# Autodesk Inventor assembly: ROBOT_1_3
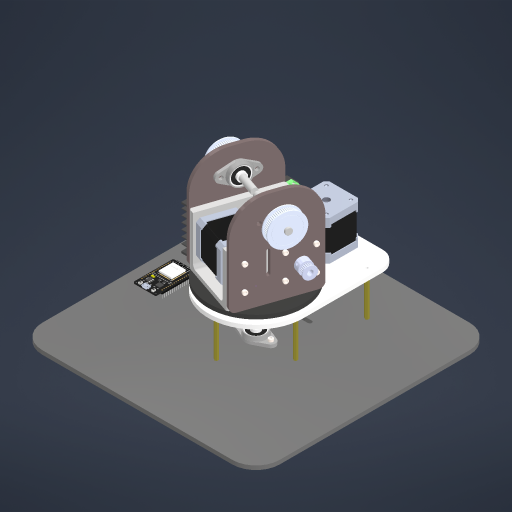
[picture p0: Inventor's stored thumbnail of the model, 512x512]
Saved by Autodesk Inventor 2023 (Build 270158000, 158)
## iProperties
Created: 2023-09-06
Part Number: ROBOT_1_3
Document SubType Name: Assembly
Designer: philo
Sending System: Autodesk Inventor 2023
Preprocessor: ST-DEVELOPER v19
Title: C:\Users\philo\OneDrive\Desktop\HK1-2024\TT ROBOT\3DVer2\ROBOT_1_2.stp
Author: philo
## Documents named in this file (23)
- C:\Users\philo\OneDrive\Desktop\HK1-2024\TT ROBOT\3DVer2\3DVer2\ROBOT_1_3.iam
- C:\Users\philo\OneDrive\Desktop\HK1-2024\TT ROBOT\3DVer2\3DVer2\DeRobot.ipt
- C:\Users\philo\OneDrive\Desktop\HK1-2024\TT ROBOT\3DVer2\3DVer2\Detron.ipt
- C:\Users\philo\OneDrive\Desktop\HK1-2024\TT ROBOT\3DVer2\3DVer2\goidoObi.ipt
- C:\Users\philo\OneDrive\Desktop\HK1-2024\TT ROBOT\3DVer2\3DVer2\truday.ipt
- C:\Users\philo\OneDrive\Desktop\HK1-2024\TT ROBOT\3DVer2\3DVer2\gt2_60teeth.iam
- C:\Users\philo\OneDrive\Desktop\HK1-2024\TT ROBOT\3DVer2\3DVer2\STEP MOTOR NEMA 17.ipt
- C:\Users\philo\OneDrive\Desktop\HK1-2024\TT ROBOT\3DVer2\3DVer2\GT2 Pulley 20 Tooth (ID6mm).ipt
- C:\Users\philo\OneDrive\Desktop\HK1-2024\TT ROBOT\3DVer2\3DVer2\M3 x 5mm.ipt
- C:\Users\philo\OneDrive\Desktop\HK1-2024\TT ROBOT\3DVer2\3DVer2\Diaquay.ipt
- C:\Users\philo\OneDrive\Desktop\HK1-2024\TT ROBOT\3DVer2\3DVer2\Tb6600.ipt
- C:\Users\philo\OneDrive\Desktop\HK1-2024\TT ROBOT\3DVer2\3DVer2\ESP-WROOM32.iam
- C:\Users\philo\OneDrive\Desktop\HK1-2024\TT ROBOT\3DVer2\3DVer2\codinhtruc.ipt
- C:\Users\philo\OneDrive\Desktop\HK1-2024\TT ROBOT\3DVer2\3DVer2\daydai.ipt
- C:\Users\philo\OneDrive\Desktop\HK1-2024\TT ROBOT\3DVer2\3DVer2\gt2smooth.ipt
- C:\Users\philo\OneDrive\Desktop\HK1-2024\TT ROBOT\3DVer2\3DVer2\trudong5mm.ipt
- C:\Users\philo\OneDrive\Desktop\HK1-2024\TT ROBOT\3DVer2\3DVer2\trucdogt2.ipt
- C:\Users\philo\OneDrive\Desktop\HK1-2024\TT ROBOT\3DVer2\3DVer2\HALL.ipt
- C:\Users\philo\OneDrive\Desktop\HK1-2024\TT ROBOT\3DVer2\3DVer2\namcham.ipt
- C:\Users\philo\OneDrive\Desktop\HK1-2024\TT ROBOT\3DVer2\3DVer2\Tamop1.ipt
- C:\Users\philo\OneDrive\Desktop\HK1-2024\TT ROBOT\3DVer2\3DVer2\60pitch pulley GT2 6mm ASSEMBLY.iam
- C:\Users\philo\OneDrive\Desktop\HK1-2024\TT ROBOT\3DVer2\3DVer2\truc8mm.ipt
- C:\Users\philo\OneDrive\Desktop\HK1-2024\TT ROBOT\3DVer2\3DVer2\giulink2.ipt
## Components (56 placed, 22 different names)
1. DeRobot:1
2. Detron:1 — Mate:33
3. goidoObi:1
4. goidoObi:2
5. truday:1 — Mate:32
6. gt2_60teeth:1 [sub-assembly]
7. STEP MOTOR NEMA 17:1
8. GT2 Pulley 20 Tooth (ID6mm):1
9. M3 x 5mm:1
10. M3 x 5mm:2
11. M3 x 5mm:3
12. M3 x 5mm:5
13. M3 x 5mm:6
14. M3 x 5mm:7
15. M3 x 5mm:8
16. Tb6600:1
17. Tb6600:2
18. ESP-WROOM32:1 [sub-assembly]
19. daydai:1
20. gt2smooth:1
21. trudong5mm:4
22. trudong5mm:5
23. trudong5mm:6
24. trudong5mm:8
25. trudong5mm:9
26. trucdogt2:1
27. HALL:1
28. M3 x 5mm:9 — Mate:38, Mate:56
29. M3 x 5mm:10 — Mate:39, Mate:58
30. M3 x 5mm:11 — Mate:37, Mate:60
31. M3 x 5mm:12 — Mate:40, Mate:57
32. M3 x 5mm:13 — Mate:41, Mate:61
33. M3 x 5mm:14 — Mate:42, Mate:59
34. M3 x 5mm:15 — Mate:43, Mate:52
35. M3 x 5mm:16 — Mate:45, Mate:51
36. M3 x 5mm:17 — Mate:46, Mate:54
37. M3 x 5mm:18 — Mate:44, Mate:50
38. M3 x 5mm:19 — Mate:47, Mate:53
39. M3 x 5mm:20 — Mate:48, Mate:55
40. gt2smooth:2 — Mate:49
41. giulink2:1 — Mate:63, Angle:3, Angle:4, Angle:5, Angle:6, Angle:7, Angle:8, Mate:64, Mate:65, Mate:67, Flush:4, Flush:5, Mate:68, Mate:69
42. Diaquay:1 — Mate:1, Mate:2, Mate:7, Mate:8, Mate:32, Mate:33, Mate:34, Angle:1, Angle:2, Flush:2, Mate:62, Flush:3, Angle:7
43. codinhtruc:2 — Mate:1, Mate:2, Mate:34, Mate:63
44. namcham:1 — Angle:2, Flush:2, Mate:62, Flush:3
45. STEP MOTOR NEMA 17:2 — Mate:27, Mate:28, Angle:6, Mate:66, Mate:67
46. STEP MOTOR NEMA 17:3 — Mate:26, Mate:30, Angle:5, Angle:8, Mate:64, Mate:65
47. Tamop1:1 — Mate:7, Mate:11, Mate:14, Mate:15, Mate:21, Flush:1, Mate:27, Mate:29, Mate:37, Mate:38, Mate:39, Mate:40, Mate:41, Mate:42, Mate:56, Mate:57, Mate:58, Mate:59, Mate:60, Mate:61, Angle:3, Mate:66, Flush:4, Mate:69
48. goidoObi:3 — Mate:11, Mate:14, Mate:15, Mate:18
49. GT2 Pulley 20 Tooth (ID6mm):2 — Mate:28, Mate:29
50. 60pitch pulley GT2 6mm ASSEMBLY:1 [sub-assembly] — Mate:21, Mate:22
51. Tamop1:2 — Mate:8, Mate:12, Mate:13, Mate:16, Mate:19, Mate:26, Mate:31, Angle:1, Mate:43, Mate:44, Mate:45, Mate:46, Mate:47, Mate:48, Mate:49, Mate:50, Mate:51, Mate:52, Mate:53, Mate:54, Mate:55, Angle:4, Flush:5, Mate:68
52. goidoObi:4 — Mate:12, Mate:13, Mate:16, Mate:17
53. GT2 Pulley 20 Tooth (ID6mm):3 — Mate:30, Mate:31
54. 60pitch pulley GT2 6mm ASSEMBLY:2 [sub-assembly] — Mate:19, Mate:20
55. truc8mm:1 — Mate:18, Mate:22, Mate:23, Flush:1
56. truc8mm:2 — Mate:17, Mate:20, Mate:23
## Relationships (72: Mate 59, Angle 8, Flush 5)
- Mate:1: Diaquay:1 ↔ codinhtruc:2
- Mate:2: Diaquay:1 ↔ codinhtruc:2
- Mate:7: Diaquay:1 ↔ Tamop1:1
- Mate:8: Diaquay:1 ↔ Tamop1:2
- Mate:11: Tamop1:1 ↔ goidoObi:3
- Mate:12: Tamop1:2 ↔ goidoObi:4
- Mate:13: Tamop1:2 ↔ goidoObi:4
- Mate:14: Tamop1:1 ↔ goidoObi:3
- Mate:15: Tamop1:1 ↔ goidoObi:3
- Mate:16: Tamop1:2 ↔ goidoObi:4
- Mate:17: goidoObi:4 ↔ truc8mm:2
- Mate:18: goidoObi:3 ↔ truc8mm:1
- Mate:19 (3 mm): Tamop1:2 ↔ 60pitch pulley GT2 6mm ASSEMBLY:2
- Mate:20: 60pitch pulley GT2 6mm ASSEMBLY:2 ↔ truc8mm:2
- Mate:21 (3 mm): Tamop1:1 ↔ 60pitch pulley GT2 6mm ASSEMBLY:1
- Mate:22: 60pitch pulley GT2 6mm ASSEMBLY:1 ↔ truc8mm:1
- Mate:23 (5 mm): truc8mm:1 ↔ truc8mm:2
- Flush:1 (-36 mm): Tamop1:1 ↔ truc8mm:1
- Mate:26: STEP MOTOR NEMA 17:3 ↔ Tamop1:2
- Mate:27: STEP MOTOR NEMA 17:2 ↔ Tamop1:1
- Mate:28: STEP MOTOR NEMA 17:2 ↔ GT2 Pulley 20 Tooth (ID6mm):2
- Mate:29 (3 mm): Tamop1:1 ↔ GT2 Pulley 20 Tooth (ID6mm):2
- Mate:30: STEP MOTOR NEMA 17:3 ↔ GT2 Pulley 20 Tooth (ID6mm):3
- Mate:31 (3 mm): Tamop1:2 ↔ GT2 Pulley 20 Tooth (ID6mm):3
- Mate:32: truday:1 ↔ Diaquay:1
- Mate:33 (6 mm): Detron:1 ↔ Diaquay:1
- Mate:34: Diaquay:1 ↔ codinhtruc:2
- Angle:1 (0 deg): Diaquay:1 ↔ Tamop1:2
- Angle:2 (0 deg): Diaquay:1 ↔ namcham:1
- Flush:2 (-60 mm): Diaquay:1 ↔ namcham:1
- Mate:37: M3 x 5mm:11 ↔ Tamop1:1
- Mate:38: M3 x 5mm:9 ↔ Tamop1:1
- Mate:39: M3 x 5mm:10 ↔ Tamop1:1
- Mate:40: M3 x 5mm:12 ↔ Tamop1:1
- Mate:41: M3 x 5mm:13 ↔ Tamop1:1
- Mate:42: M3 x 5mm:14 ↔ Tamop1:1
- Mate:43: M3 x 5mm:15 ↔ Tamop1:2
- Mate:44: M3 x 5mm:18 ↔ Tamop1:2
- Mate:45: M3 x 5mm:16 ↔ Tamop1:2
- Mate:46: M3 x 5mm:17 ↔ Tamop1:2
- Mate:47: M3 x 5mm:19 ↔ Tamop1:2
- Mate:48: M3 x 5mm:20 ↔ Tamop1:2
- Mate:49 (8 mm): gt2smooth:2 ↔ Tamop1:2
- Mate:50: M3 x 5mm:18 ↔ Tamop1:2
- Mate:51: M3 x 5mm:16 ↔ Tamop1:2
- Mate:52: M3 x 5mm:15 ↔ Tamop1:2
- Mate:53: M3 x 5mm:19 ↔ Tamop1:2
- Mate:54: M3 x 5mm:17 ↔ Tamop1:2
- Mate:55: M3 x 5mm:20 ↔ Tamop1:2
- Mate:56: M3 x 5mm:9 ↔ Tamop1:1
- Mate:57: M3 x 5mm:12 ↔ Tamop1:1
- Mate:58: M3 x 5mm:10 ↔ Tamop1:1
- Mate:59: M3 x 5mm:14 ↔ Tamop1:1
- Mate:60: M3 x 5mm:11 ↔ Tamop1:1
- Mate:61: M3 x 5mm:13 ↔ Tamop1:1
- Mate:62 (-3 mm): Diaquay:1 ↔ namcham:1
- Flush:3: Diaquay:1 ↔ namcham:1
- Mate:63: giulink2:1 ↔ codinhtruc:2
- Angle:3 (90 deg): giulink2:1 ↔ Tamop1:1
- Angle:4 (90 deg): giulink2:1 ↔ Tamop1:2
- Angle:5 (0 deg): giulink2:1 ↔ STEP MOTOR NEMA 17:3
- Angle:6 (0 deg): giulink2:1 ↔ STEP MOTOR NEMA 17:2
- Angle:7 (90 deg): giulink2:1 ↔ Diaquay:1
- Angle:8 (0 deg): giulink2:1 ↔ STEP MOTOR NEMA 17:3
- Mate:64: giulink2:1 ↔ STEP MOTOR NEMA 17:3
- Mate:65: giulink2:1 ↔ STEP MOTOR NEMA 17:3
- Mate:66: STEP MOTOR NEMA 17:2 ↔ Tamop1:1
- Mate:67: giulink2:1 ↔ STEP MOTOR NEMA 17:2
- Flush:4: giulink2:1 ↔ Tamop1:1
- Flush:5: giulink2:1 ↔ Tamop1:2
- Mate:68: giulink2:1 ↔ Tamop1:2
- Mate:69: giulink2:1 ↔ Tamop1:1
